# Autodesk Inventor assembly: パネル型スカラアームMISUMIアルミフレーム作成Ver
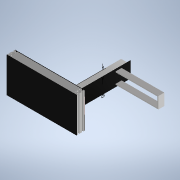
[picture p0: Inventor's stored thumbnail of the model, 180x180]
Saved by Autodesk Inventor 2022 (Build 260153000, 153)
## iProperties
Created: 2022-12-05
Part Number: パネル型スカラアームMISUMIアルミフレーム作成Ver
Document SubType Name: Assembly
Designer: tdn82
Author: tdn82
## Documents named in this file (16)
- C:\Users\tdn82\OneDrive\ドキュメント\Inventor\卒業研究パネル型スカラアーム\GrabCAD\panel-type-scalar-arm\パネル型スカラアーム\パネル型スカラアームMISUMIアルミフレーム作成Ver.iam
- C:\Users\tdn82\OneDrive\ドキュメント\Inventor\卒業研究パネル型スカラアーム\GrabCAD\panel-type-scalar-arm\パネル型スカラアーム\HFSF5-2040-180-LWH-RWH.ipt
- C:\Users\tdn82\OneDrive\ドキュメント\Inventor\卒業研究パネル型スカラアーム\GrabCAD\panel-type-scalar-arm\パネル型スカラアーム\HFSF5-2040-320-TPW.ipt
- C:\Users\tdn82\OneDrive\ドキュメント\Inventor\卒業研究パネル型スカラアーム\GrabCAD\panel-type-scalar-arm\パネル型スカラアーム\後ろカバー.ipt
- C:\Users\tdn82\OneDrive\ドキュメント\Inventor\卒業研究パネル型スカラアーム\GrabCAD\panel-type-scalar-arm\パネル型スカラアーム\サーボモータ固定用１軸目.ipt
- C:\Users\tdn82\OneDrive\ドキュメント\Inventor\卒業研究パネル型スカラアーム\GrabCAD\panel-type-scalar-arm\パネル型スカラアーム\サーボモータB3M-SC-1170-AB3M1100_scale.ipt
- C:\Users\tdn82\OneDrive\ドキュメント\Inventor\卒業研究パネル型スカラアーム\GrabCAD\panel-type-scalar-arm\パネル型スカラアーム\サーボ固定パーツ３Dプリンタ出力実験\サーボモータ固定用２軸目3mm改.ipt
- C:\Users\tdn82\OneDrive\ドキュメント\Inventor\卒業研究パネル型スカラアーム\GrabCAD\panel-type-scalar-arm\パネル型スカラアーム\横長2ndフラットバー上 アルミフレーム用.ipt
- C:\Users\tdn82\OneDrive\ドキュメント\Inventor\卒業研究パネル型スカラアーム\GrabCAD\panel-type-scalar-arm\パネル型スカラアーム\前カバー中盤左アーム固定.ipt
- C:\Users\tdn82\OneDrive\ドキュメント\Inventor\卒業研究パネル型スカラアーム\GrabCAD\panel-type-scalar-arm\パネル型スカラアーム\アルミフリーホーン02137_AluminumFreeHornWithBearing_B3M_6000.ipt
- C:\Users\tdn82\OneDrive\ドキュメント\Inventor\卒業研究パネル型スカラアーム\GrabCAD\panel-type-scalar-arm\パネル型スカラアーム\横長3rdフラットバー下.ipt
- C:\Users\tdn82\OneDrive\ドキュメント\Inventor\卒業研究パネル型スカラアーム\GrabCAD\panel-type-scalar-arm\パネル型スカラアーム\縦長3rdフラットバー.ipt
- C:\Users\tdn82\OneDrive\ドキュメント\Inventor\卒業研究パネル型スカラアーム\GrabCAD\panel-type-scalar-arm\パネル型スカラアーム\横長2ndフラットバー下 アルミフレーム用.ipt
- C:\Users\tdn82\OneDrive\ドキュメント\Inventor\卒業研究パネル型スカラアーム\GrabCAD\panel-type-scalar-arm\パネル型スカラアーム\前カバー中段右.ipt
- C:\Users\tdn82\OneDrive\ドキュメント\Inventor\卒業研究パネル型スカラアーム\GrabCAD\panel-type-scalar-arm\パネル型スカラアーム\前上カバーサーボ隠し.ipt
- C:\Users\tdn82\OneDrive\ドキュメント\Inventor\卒業研究パネル型スカラアーム\GrabCAD\panel-type-scalar-arm\パネル型スカラアーム\前下カバーサーボ隠し.ipt
## Components (19 placed, 15 different names)
1. HFSF5-2040-180-LWH-RWH:1 — 挿入:6, 挿入:8, 挿入:9, 挿入:10
2. HFSF5-2040-180-LWH-RWH:2 — 挿入:5, 挿入:7, メイト:2, メイト:4, フラッシュ:1, メイト:12, メイト:14
3. HFSF5-2040-320-TPW:1 — 挿入:5, 挿入:6, 挿入:7, 挿入:8, メイト:1, メイト:5, メイト:13
4. HFSF5-2040-320-TPW:2 — 挿入:9, 挿入:10, メイト:3
5. 後ろカバー:1 — メイト:1, メイト:2, メイト:3, 角度:2, 角度:3
6. サーボモータ固定用１軸目:1 — 挿入:11, 挿入:12, 挿入:13, メイト:4, フラッシュ:1
7. サーボモータB3M-SC-1170-AB3M1100_scale:1 — 挿入:11, 挿入:12, 挿入:13, メイト:5, 挿入:14
8. サーボモータ固定用２軸目3mm改:1 — 挿入:15, 挿入:16, 挿入:18, 挿入:19
9. 横長2ndフラットバー上 アルミフレーム用:1 — 挿入:14, メイト:7, フラッシュ:3, 角度:3, メイト:19
10. 前カバー中盤左アーム固定:1 — メイト:7, 挿入:15, 挿入:16, 挿入:23, 挿入:24, フラッシュ:3, メイト:19
11. サーボモータB3M-SC-1170-AB3M1100_scale:2 — 挿入:17, 挿入:18, 挿入:19, 挿入:20
12. アルミフリーホーン02137_AluminumFreeHornWithBearing_B3M_6000:1 — 挿入:17, 挿入:21, 挿入:22
13. 横長3rdフラットバー下:1 — 挿入:20, フラッシュ:2, メイト:9, メイト:10
14. 横長3rdフラットバー下:2 — 挿入:21, 挿入:22, フラッシュ:2, メイト:8, 角度:2
15. 縦長3rdフラットバー:1 — メイト:8, メイト:9, メイト:10
16. 横長2ndフラットバー下 アルミフレーム用:1 — 挿入:23, 挿入:24
17. 前カバー中段右:1 — メイト:12, メイト:15, メイト:16, メイト:17, メイト:18
18. 前上カバーサーボ隠し:1 — メイト:13, メイト:14, メイト:15, メイト:16
19. 前下カバーサーボ隠し:1 — メイト:17, メイト:18
## Relationships (42: Insert 20, Mate 17, Flush 3, Angle 2)
- 挿入:5 [Insert]: HFSF5-2040-180-LWH-RWH:2 ↔ HFSF5-2040-320-TPW:1
- 挿入:6 [Insert]: HFSF5-2040-180-LWH-RWH:1 ↔ HFSF5-2040-320-TPW:1
- 挿入:7 [Insert]: HFSF5-2040-180-LWH-RWH:2 ↔ HFSF5-2040-320-TPW:1
- 挿入:8 [Insert]: HFSF5-2040-180-LWH-RWH:1 ↔ HFSF5-2040-320-TPW:1
- 挿入:9 [Insert]: HFSF5-2040-180-LWH-RWH:1 ↔ HFSF5-2040-320-TPW:2
- 挿入:10 [Insert]: HFSF5-2040-180-LWH-RWH:1 ↔ HFSF5-2040-320-TPW:2
- メイト:1 [Mate]: HFSF5-2040-320-TPW:1 ↔ 後ろカバー:1
- メイト:2 [Mate] (1 mm): HFSF5-2040-180-LWH-RWH:2 ↔ 後ろカバー:1
- メイト:3 [Mate] (1 mm): HFSF5-2040-320-TPW:2 ↔ 後ろカバー:1
- 挿入:11 [Insert]: サーボモータ固定用１軸目:1 ↔ サーボモータB3M-SC-1170-AB3M1100_scale:1
- 挿入:12 [Insert]: サーボモータ固定用１軸目:1 ↔ サーボモータB3M-SC-1170-AB3M1100_scale:1
- 挿入:13 [Insert]: サーボモータ固定用１軸目:1 ↔ サーボモータB3M-SC-1170-AB3M1100_scale:1
- メイト:4 [Mate]: HFSF5-2040-180-LWH-RWH:2 ↔ サーボモータ固定用１軸目:1
- フラッシュ:1 [Flush]: HFSF5-2040-180-LWH-RWH:2 ↔ サーボモータ固定用１軸目:1
- メイト:5 [Mate] (0.5 mm): HFSF5-2040-320-TPW:1 ↔ サーボモータB3M-SC-1170-AB3M1100_scale:1
- 挿入:14 [Insert]: サーボモータB3M-SC-1170-AB3M1100_scale:1 ↔ 横長2ndフラットバー上 アルミフレーム用:1
- メイト:7 [Mate]: 横長2ndフラットバー上 アルミフレーム用:1 ↔ 前カバー中盤左アーム固定:1
- 挿入:15 [Insert]: サーボモータ固定用２軸目3mm改:1 ↔ 前カバー中盤左アーム固定:1
- 挿入:16 [Insert]: サーボモータ固定用２軸目3mm改:1 ↔ 前カバー中盤左アーム固定:1
- 挿入:17 [Insert]: サーボモータB3M-SC-1170-AB3M1100_scale:2 ↔ アルミフリーホーン02137_AluminumFreeHornWithBearing_B3M_6000:1
- 挿入:18 [Insert]: サーボモータ固定用２軸目3mm改:1 ↔ サーボモータB3M-SC-1170-AB3M1100_scale:2
- 挿入:19 [Insert]: サーボモータ固定用２軸目3mm改:1 ↔ サーボモータB3M-SC-1170-AB3M1100_scale:2
- 挿入:20 [Insert]: サーボモータB3M-SC-1170-AB3M1100_scale:2 ↔ 横長3rdフラットバー下:1
- 挿入:21 [Insert]: アルミフリーホーン02137_AluminumFreeHornWithBearing_B3M_6000:1 ↔ 横長3rdフラットバー下:2
- 挿入:22 [Insert]: アルミフリーホーン02137_AluminumFreeHornWithBearing_B3M_6000:1 ↔ 横長3rdフラットバー下:2
- フラッシュ:2 [Flush]: 横長3rdフラットバー下:1 ↔ 横長3rdフラットバー下:2
- メイト:8 [Mate]: 横長3rdフラットバー下:2 ↔ 縦長3rdフラットバー:1
- メイト:9 [Mate]: 横長3rdフラットバー下:1 ↔ 縦長3rdフラットバー:1
- メイト:10 [Mate]: 横長3rdフラットバー下:1 ↔ 縦長3rdフラットバー:1
- 角度:2 [Angle] (0 deg): 後ろカバー:1 ↔ 横長3rdフラットバー下:2
- 挿入:23 [Insert]: 前カバー中盤左アーム固定:1 ↔ 横長2ndフラットバー下 アルミフレーム用:1
- 挿入:24 [Insert]: 前カバー中盤左アーム固定:1 ↔ 横長2ndフラットバー下 アルミフレーム用:1
- メイト:12 [Mate]: HFSF5-2040-180-LWH-RWH:2 ↔ 前カバー中段右:1
- メイト:13 [Mate] (-1 mm): HFSF5-2040-320-TPW:1 ↔ 前上カバーサーボ隠し:1
- メイト:14 [Mate] (-1 mm): HFSF5-2040-180-LWH-RWH:2 ↔ 前上カバーサーボ隠し:1
- メイト:15 [Mate]: 前カバー中段右:1 ↔ 前上カバーサーボ隠し:1
- メイト:16 [Mate]: 前カバー中段右:1 ↔ 前上カバーサーボ隠し:1
- メイト:17 [Mate]: 前カバー中段右:1 ↔ 前下カバーサーボ隠し:1
- メイト:18 [Mate]: 前カバー中段右:1 ↔ 前下カバーサーボ隠し:1
- フラッシュ:3 [Flush] (29 mm): 横長2ndフラットバー上 アルミフレーム用:1 ↔ 前カバー中盤左アーム固定:1
- 角度:3 [Angle] (90 deg): 後ろカバー:1 ↔ 横長2ndフラットバー上 アルミフレーム用:1
- メイト:19 [Mate]: 横長2ndフラットバー上 アルミフレーム用:1 ↔ 前カバー中盤左アーム固定:1
